# Autodesk Inventor assembly: Assemblies_Cradle
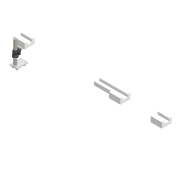
[picture p0: Inventor's stored thumbnail of the model, 180x180]
Saved by Autodesk Inventor 2021 (Build 250183000, 183)
## iProperties
Created: 2021-10-08
Part Number: Assemblies_Cradle
Document SubType Name: Assembly
Designer: Rik Ubaghs
Author: Rik Ubaghs
## Documents named in this file (10)
- C:\Users\Rik Ubaghs\Documents\git\git_upload\open_mrcradle_mouse_mk1\production\ipt\assemblies\assemblies_rails.iam
- C:\Users\Rik Ubaghs\Documents\git\git_upload\open_mrcradle_mouse_mk1\production\ipt\cradle\cradle_slide_front_mk1.ipt
- C:\Users\Rik Ubaghs\Documents\git\git_upload\open_mrcradle_mouse_mk1\production\ipt\cradle\cradle_slidebase_mk1.ipt
- C:\Users\Rik Ubaghs\Documents\git\git_upload\open_mrcradle_mouse_mk1\production\ipt\cradle\cradle_av4m_ext.ipt
- C:\Users\Rik Ubaghs\Documents\git\git_upload\open_mrcradle_mouse_mk1\production\ipt\cradle\cradle_c1515m_ext.ipt
- C:\Users\Rik Ubaghs\Documents\git\git_upload\open_mrcradle_mouse_mk1\production\ipt\cradle\cradle_mb1015m_ext.ipt
- C:\Users\Rik Ubaghs\Documents\git\git_upload\open_mrcradle_mouse_mk1\production\ipt\cradle\cradle_p300m_ext.ipt
- C:\Users\Rik Ubaghs\Documents\git\git_upload\open_mrcradle_mouse_mk1\production\ipt\cradle\cradle_pb4m_ext.ipt
- C:\Users\Rik Ubaghs\Documents\git\git_upload\open_mrcradle_mouse_mk1\production\ipt\cradle\cradle_slide_back_mk1.ipt
- C:\Users\Rik Ubaghs\Documents\git\git_upload\open_mrcradle_mouse_mk1\production\ipt\cradle\cradle_psham_ext.ipt
## Components (15 placed, 9 different names)
1. cradle_av4m_ext:1 — Mate:35, Mate:38
2. cradle_av4m_ext:2 — Mate:31, Mate:34
3. cradle_av4m_ext:3 — Mate:36, Mate:37
4. cradle_av4m_ext:4 — Mate:32, Mate:33
5. cradle_pb4m_ext:1 — Mate:29, Mate:30, Mate:45, Tangent:4, Tangent:5, Mate:54
6. cradle_c1515m_ext:1 — Mate:40, Angle:5, Tangent:3, Mate:44, Angle:6, Flush:2, Mate:52
7. cradle_mb1015m_ext:1 — Mate:30, Mate:31, Mate:32, Mate:33, Mate:34, Mate:35, Mate:36, Mate:37, Mate:38, Angle:5, Tangent:4, Tangent:5
8. cradle_mb1015m_ext:2 — Tangent:3, Mate:44, Angle:6, Flush:2, Mate:51, Flush:8, Flush:9
9. cradle_p300m_ext:1 — Mate:29, Mate:40, Mate:45, Mate:53
10. cradle_psham_ext:1 — Mate:52, Mate:53, Mate:54
11. cradle_slidebase_mk1:1 — Mate:22, Mate:23, Mate:24, Flush:5
12. cradle_slidebase_mk1:2 — Mate:25, Mate:26, Mate:27, Flush:5
13. cradle_slide_back_mk1:1 — Flush:6, Flush:7, Mate:51, Flush:8, Flush:9
14. cradle_slide_back_mk1:2 — Mate:22, Mate:23, Mate:24, Flush:4, Mate:49, Flush:6, Flush:7
15. cradle_slide_front_mk1:1 — Mate:25, Mate:26, Mate:27, Flush:4, Mate:49
## Relationships (36: Mate 24, Flush 7, Tangent 3, Angle 2)
- Mate:22: cradle_slidebase_mk1:1 ↔ cradle_slide_back_mk1:2
- Mate:23: cradle_slidebase_mk1:1 ↔ cradle_slide_back_mk1:2
- Mate:24: cradle_slidebase_mk1:1 ↔ cradle_slide_back_mk1:2
- Mate:25: cradle_slidebase_mk1:2 ↔ cradle_slide_front_mk1:1
- Mate:26: cradle_slidebase_mk1:2 ↔ cradle_slide_front_mk1:1
- Mate:27: cradle_slidebase_mk1:2 ↔ cradle_slide_front_mk1:1
- Mate:29: cradle_pb4m_ext:1 ↔ cradle_p300m_ext:1
- Mate:30: cradle_pb4m_ext:1 ↔ cradle_mb1015m_ext:1
- Mate:31: cradle_av4m_ext:2 ↔ cradle_mb1015m_ext:1
- Mate:32: cradle_av4m_ext:4 ↔ cradle_mb1015m_ext:1
- Mate:33: cradle_av4m_ext:4 ↔ cradle_mb1015m_ext:1
- Mate:34: cradle_av4m_ext:2 ↔ cradle_mb1015m_ext:1
- Mate:35: cradle_av4m_ext:1 ↔ cradle_mb1015m_ext:1
- Mate:36: cradle_av4m_ext:3 ↔ cradle_mb1015m_ext:1
- Mate:37: cradle_av4m_ext:3 ↔ cradle_mb1015m_ext:1
- Mate:38: cradle_av4m_ext:1 ↔ cradle_mb1015m_ext:1
- Mate:40: cradle_c1515m_ext:1 ↔ cradle_p300m_ext:1
- Angle:5 (0 deg): cradle_c1515m_ext:1 ↔ cradle_mb1015m_ext:1
- Tangent:3: cradle_c1515m_ext:1 ↔ cradle_mb1015m_ext:2
- Mate:44: cradle_c1515m_ext:1 ↔ cradle_mb1015m_ext:2
- Angle:6 (0 deg): cradle_c1515m_ext:1 ↔ cradle_mb1015m_ext:2
- Flush:2 (-10 mm): cradle_c1515m_ext:1 ↔ cradle_mb1015m_ext:2
- Mate:45: cradle_pb4m_ext:1 ↔ cradle_p300m_ext:1
- Tangent:4 (2 mm): cradle_pb4m_ext:1 ↔ cradle_mb1015m_ext:1
- Tangent:5 (27 mm): cradle_pb4m_ext:1 ↔ cradle_mb1015m_ext:1
- Flush:4: cradle_slide_back_mk1:2 ↔ cradle_slide_front_mk1:1
- Flush:5: cradle_slidebase_mk1:1 ↔ cradle_slidebase_mk1:2
- Mate:49 (400 mm): cradle_slide_back_mk1:2 ↔ cradle_slide_front_mk1:1
- Flush:6: cradle_slide_back_mk1:1 ↔ cradle_slide_back_mk1:2
- Flush:7: cradle_slide_back_mk1:1 ↔ cradle_slide_back_mk1:2
- Mate:51: cradle_mb1015m_ext:2 ↔ cradle_slide_back_mk1:1
- Flush:8 (-10 mm): cradle_mb1015m_ext:2 ↔ cradle_slide_back_mk1:1
- Flush:9 (20 mm): cradle_mb1015m_ext:2 ↔ cradle_slide_back_mk1:1
- Mate:52: cradle_c1515m_ext:1 ↔ cradle_psham_ext:1
- Mate:53: cradle_p300m_ext:1 ↔ cradle_psham_ext:1
- Mate:54: cradle_pb4m_ext:1 ↔ cradle_psham_ext:1
